# Autodesk Inventor assembly: bpSupAssy37
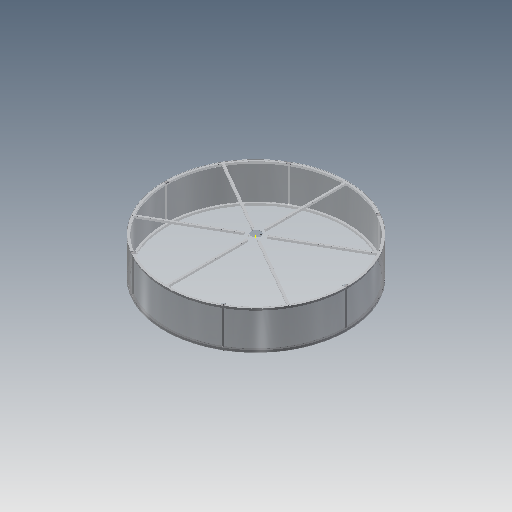
[picture p0: Inventor's stored thumbnail of the model, 512x512]
Saved by Autodesk Inventor 2017 (Build 210142000, 142)
## iProperties
Created: 2016-10-11
Part Number: bpSupAssy37
Document SubType Name: Assembly
Designer: krosie
Author: krosie
## Documents named in this file (10)
- C:\Users\krosie\Google Drive\HERA\hera-cad\feed\bpSupAssy37\bpSupAssy37.iam
- C:\Users\krosie\Google Drive\HERA\hera-cad\jigs\bpSparJig.ipt
- C:\Users\krosie\Google Drive\HERA\hera-cad\feed\bpSupAssy37\FeedHoop37.ipt
- C:\Users\krosie\Google Drive\HERA\hera-cad\feed\bpSupAssy37\bpSupArm37.ipt
- C:\Users\krosie\Google Drive\HERA\hera-cad\feed\bpSupAssy37\bpSupVertArm37.ipt
- C:\Users\krosie\Google Drive\HERA\hera-cad\feed\bpSupAssy37\FlatTee.ipt
- C:\Users\krosie\Google Drive\HERA\hera-cad\feed\bpCylinder.ipt
- C:\Users\krosie\Google Drive\HERA\hera-cad\feed\bpScreen.ipt
- C:\Users\krosie\Documents\Inventor\Content Center Files\R2017\en-US\ANSI B 18.2.4.1 M(1)\ANSI B 18.2.4.1 M - M8 x 1.25Style 1.ipt
- C:\Users\krosie\Documents\Inventor\Content Center Files\R2017\en-US\AS 1427(05)\AS 1427 - M5 x 12(5) II.ipt
## Components (50 placed, 9 different names)
1. bpSparJig:1 — Flush:1, Flush:2, Mate:1, Mate:3, Mate:14, Mate:15, Mate:17, Mate:21, Mate:23
2. FeedHoop37:1 — Mate:1, Mate:3, Mate:4, Mate:5, Mate:6, Insert:1, Mate:15, Tangent:1, Mate:19, Mate:20, Mate:22, Mate:48, Mate:49, Mate:54, Mate:55, Mate:59, Mate:61, Mate:62, Mate:65, Mate:66, Mate:67, Mate:68, Mate:69
3. FeedHoop37:2 — Mate:16, Mate:17, Mate:18, Mate:19, Mate:50, Mate:51, Mate:52, Mate:53, Mate:56, Mate:57, Mate:58, Mate:60, Mate:63, Mate:64, Mate:70, Mate:71
4. bpCylinder:1 — Mate:14, Mate:20
5. bpScreen:1 — Mate:21, Mate:22, Mate:23
6. AS 1427 H - Metric M5 x 12:1
7. AS 1427 H - Metric M5 x 12:2
8. AS 1427 H - Metric M5 x 12:3
9. Hex Nut Metric M8 x 1.25:1 — Mate:24, Mate:66
10. Hex Nut Metric M8 x 1.25:2 — Mate:25, Mate:67
11. Hex Nut Metric M8 x 1.25:3 — Mate:42, Mate:71
12. Hex Nut Metric M8 x 1.25:4 — Mate:43, Mate:70
13. Hex Nut Metric M8 x 1.25:5 — Mate:36, Mate:50
14. Hex Nut Metric M8 x 1.25:6 — Mate:37, Mate:51
15. Hex Nut Metric M8 x 1.25:7 — Mate:40, Mate:64
16. Hex Nut Metric M8 x 1.25:8 — Mate:41, Mate:63
17. Hex Nut Metric M8 x 1.25:9 — Mate:45, Mate:54
18. Hex Nut Metric M8 x 1.25:10 — Mate:44, Mate:55
19. Hex Nut Metric M8 x 1.25:11 — Mate:34, Mate:53
20. Hex Nut Metric M8 x 1.25:12 — Mate:35, Mate:52
21. Hex Nut Metric M8 x 1.25:13 — Mate:39, Mate:57
22. Hex Nut Metric M8 x 1.25:14 — Mate:38, Mate:56
23. Hex Nut Metric M8 x 1.25:15 — Mate:26, Mate:68
24. Hex Nut Metric M8 x 1.25:16 — Mate:27, Mate:69
25. Hex Nut Metric M8 x 1.25:17 — Mate:29, Mate:58
26. Hex Nut Metric M8 x 1.25:18 — Mate:28, Mate:60
27. Hex Nut Metric M8 x 1.25:19 — Mate:30, Mate:61
28. Hex Nut Metric M8 x 1.25:20 — Mate:31, Mate:59
29. Hex Nut Metric M8 x 1.25:21 — Mate:32, Mate:62
30. Hex Nut Metric M8 x 1.25:22 — Mate:33, Mate:65
31. Hex Nut Metric M8 x 1.25:23 — Mate:46, Mate:49
32. Hex Nut Metric M8 x 1.25:24 — Mate:47, Mate:48
33. FlatTee:1 — Mate:6, Mate:8, Tangent:1
34. bpSupVertArm37:1 — Insert:1, Mate:32, Mate:33, Mate:40, Mate:41
35. bpSupArm37:1 — Mate:4, Mate:5, Mate:8
36. FlatTee:2
37. bpSupVertArm37:2 — Mate:28, Mate:29, Mate:30, Mate:31
38. bpSupArm37:2
39. FlatTee:3
40. bpSupVertArm37:3 — Mate:26, Mate:27, Mate:38, Mate:39
41. bpSupArm37:3
42. FlatTee:4
43. bpSupVertArm37:4 — Mate:34, Mate:35, Mate:44, Mate:45
44. bpSupArm37:4
45. FlatTee:5
46. bpSupVertArm37:5 — Mate:18, Mate:36, Mate:37, Mate:46, Mate:47
47. bpSupArm37:5
48. FlatTee:6
49. bpSupVertArm37:6 — Mate:16, Mate:24, Mate:25, Mate:42, Mate:43
50. bpSupArm37:6
## Component patterns: (6 elements, first: FlatTee:1 + bpSupVertArm37:1 + bpSupArm37:1)
## Relationships (68: Mate 64, Flush 2, Insert 1, Tangent 1)
- Flush:1: bpSparJig:1
- Flush:2: bpSparJig:1
- Mate:1: bpSparJig:1 ↔ FeedHoop37:1
- Mate:3: bpSparJig:1 ↔ FeedHoop37:1
- Mate:4: FeedHoop37:1 ↔ bpSupArm37:1
- Mate:5: FeedHoop37:1 ↔ bpSupArm37:1
- Mate:6: FeedHoop37:1 ↔ FlatTee:1
- Mate:8: FlatTee:1 ↔ bpSupArm37:1
- Mate:14: bpSparJig:1 ↔ bpCylinder:1
- Insert:1 (-367 mm): FeedHoop37:1 ↔ bpSupVertArm37:1
- Mate:15: bpSparJig:1 ↔ FeedHoop37:1
- Tangent:1: FeedHoop37:1 ↔ FlatTee:1
- Mate:16: FeedHoop37:2 ↔ bpSupVertArm37:6
- Mate:17: bpSparJig:1 ↔ FeedHoop37:2
- Mate:18: FeedHoop37:2 ↔ bpSupVertArm37:5
- Mate:19 (-360 mm): FeedHoop37:1 ↔ FeedHoop37:2
- Mate:20: FeedHoop37:1 ↔ bpCylinder:1
- Mate:21: bpSparJig:1 ↔ bpScreen:1
- Mate:22: FeedHoop37:1 ↔ bpScreen:1
- Mate:23: bpSparJig:1 ↔ bpScreen:1
- Mate:24: Hex Nut Metric M8 x 1.25:1 ↔ bpSupVertArm37:6
- Mate:25: Hex Nut Metric M8 x 1.25:2 ↔ bpSupVertArm37:6
- Mate:26: Hex Nut Metric M8 x 1.25:15 ↔ bpSupVertArm37:3
- Mate:27: Hex Nut Metric M8 x 1.25:16 ↔ bpSupVertArm37:3
- Mate:28: Hex Nut Metric M8 x 1.25:18 ↔ bpSupVertArm37:2
- Mate:29: Hex Nut Metric M8 x 1.25:17 ↔ bpSupVertArm37:2
- Mate:30: Hex Nut Metric M8 x 1.25:19 ↔ bpSupVertArm37:2
- Mate:31: Hex Nut Metric M8 x 1.25:20 ↔ bpSupVertArm37:2
- Mate:32: Hex Nut Metric M8 x 1.25:21 ↔ bpSupVertArm37:1
- Mate:33: Hex Nut Metric M8 x 1.25:22 ↔ bpSupVertArm37:1
- Mate:34: Hex Nut Metric M8 x 1.25:11 ↔ bpSupVertArm37:4
- Mate:35: Hex Nut Metric M8 x 1.25:12 ↔ bpSupVertArm37:4
- Mate:36: Hex Nut Metric M8 x 1.25:5 ↔ bpSupVertArm37:5
- Mate:37: Hex Nut Metric M8 x 1.25:6 ↔ bpSupVertArm37:5
- Mate:38: Hex Nut Metric M8 x 1.25:14 ↔ bpSupVertArm37:3
- Mate:39: Hex Nut Metric M8 x 1.25:13 ↔ bpSupVertArm37:3
- Mate:40: Hex Nut Metric M8 x 1.25:7 ↔ bpSupVertArm37:1
- Mate:41: Hex Nut Metric M8 x 1.25:8 ↔ bpSupVertArm37:1
- Mate:42: Hex Nut Metric M8 x 1.25:3 ↔ bpSupVertArm37:6
- Mate:43: Hex Nut Metric M8 x 1.25:4 ↔ bpSupVertArm37:6
- Mate:44: Hex Nut Metric M8 x 1.25:10 ↔ bpSupVertArm37:4
- Mate:45: Hex Nut Metric M8 x 1.25:9 ↔ bpSupVertArm37:4
- Mate:46: Hex Nut Metric M8 x 1.25:23 ↔ bpSupVertArm37:5
- Mate:47: Hex Nut Metric M8 x 1.25:24 ↔ bpSupVertArm37:5
- Mate:48: FeedHoop37:1 ↔ Hex Nut Metric M8 x 1.25:24
- Mate:49: FeedHoop37:1 ↔ Hex Nut Metric M8 x 1.25:23
- Mate:50: FeedHoop37:2 ↔ Hex Nut Metric M8 x 1.25:5
- Mate:51: FeedHoop37:2 ↔ Hex Nut Metric M8 x 1.25:6
- Mate:52: FeedHoop37:2 ↔ Hex Nut Metric M8 x 1.25:12
- Mate:53: FeedHoop37:2 ↔ Hex Nut Metric M8 x 1.25:11
- Mate:54: FeedHoop37:1 ↔ Hex Nut Metric M8 x 1.25:9
- Mate:55: FeedHoop37:1 ↔ Hex Nut Metric M8 x 1.25:10
- Mate:56: FeedHoop37:2 ↔ Hex Nut Metric M8 x 1.25:14
- Mate:57: FeedHoop37:2 ↔ Hex Nut Metric M8 x 1.25:13
- Mate:58: FeedHoop37:2 ↔ Hex Nut Metric M8 x 1.25:17
- Mate:59: FeedHoop37:1 ↔ Hex Nut Metric M8 x 1.25:20
- Mate:60: FeedHoop37:2 ↔ Hex Nut Metric M8 x 1.25:18
- Mate:61: FeedHoop37:1 ↔ Hex Nut Metric M8 x 1.25:19
- Mate:62: FeedHoop37:1 ↔ Hex Nut Metric M8 x 1.25:21
- Mate:63: FeedHoop37:2 ↔ Hex Nut Metric M8 x 1.25:8
- Mate:64: FeedHoop37:2 ↔ Hex Nut Metric M8 x 1.25:7
- Mate:65: FeedHoop37:1 ↔ Hex Nut Metric M8 x 1.25:22
- Mate:66: FeedHoop37:1 ↔ Hex Nut Metric M8 x 1.25:1
- Mate:67: FeedHoop37:1 ↔ Hex Nut Metric M8 x 1.25:2
- Mate:68: FeedHoop37:1 ↔ Hex Nut Metric M8 x 1.25:15
- Mate:69: FeedHoop37:1 ↔ Hex Nut Metric M8 x 1.25:16
- Mate:70: FeedHoop37:2 ↔ Hex Nut Metric M8 x 1.25:4
- Mate:71: FeedHoop37:2 ↔ Hex Nut Metric M8 x 1.25:3
